# Autodesk Inventor assembly: Hinge
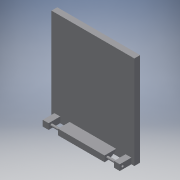
[picture p0: Inventor's stored thumbnail of the model, 180x180]
Saved by Autodesk Inventor 2016 (Build 200138000, 138)
## iProperties
Created: 2017-02-17
Part Number: Hinge
Document SubType Name: Assembly
Designer: RoboticsUser
Author: RoboticsUser
## Documents named in this file (3)
- C:\Robotics\CAD\2016-17_CAD\Hinge.iam
- C:\Robotics\CAD\2016-17_CAD\HingPartUno.ipt
- C:\Robotics\CAD\2016-17_CAD\HingPart2.ipt
## Components (2 placed, 2 different names)
1. HingPartUno:1 — Mate:1, Flush:1, Flush:2, Mate:2
2. HingPart2:1 — Mate:1, Flush:1, Flush:2, Mate:2
## Relationships (4: Mate 2, Flush 2)
- Mate:1: HingPartUno:1 ↔ HingPart2:1
- Flush:1: HingPartUno:1 ↔ HingPart2:1
- Flush:2: HingPartUno:1 ↔ HingPart2:1
- Mate:2 (5.1308 mm): HingPartUno:1 ↔ HingPart2:1
